# Autodesk Inventor assembly: Gripper Assembly
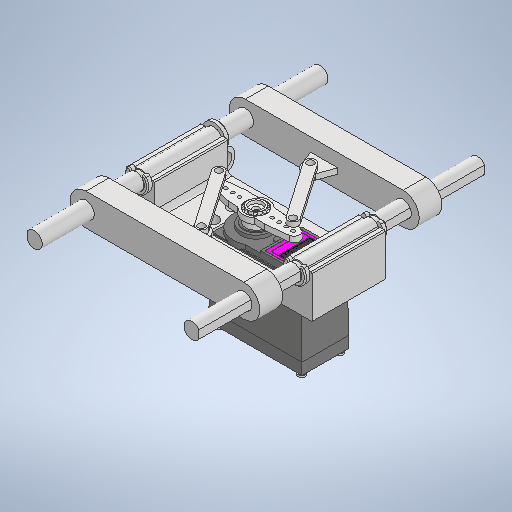
[picture p0: Inventor's stored thumbnail of the model, 512x512]
Saved by Autodesk Inventor 2025.2 (Build 292293000, 293)
## iProperties
Created: 2025-01-12
Part Number: Gripper Assembly
Document SubType Name: Assembly
Designer: caomi
Author: caomi
## Documents named in this file (8)
- C:\mnguyen\H2A\cad\Gripper\Gripper Assembly.iam
- C:\mnguyen\H2A\cad\Gripper\mg996R_v2\mg996R_v2\mg996R_v2.ipt
- C:\mnguyen\H2A\cad\Gripper\Servo mount - front.ipt
- C:\mnguyen\H2A\cad\Gripper\Linear Rod.ipt
- C:\mnguyen\H2A\cad\Gripper\Gripper_arms.ipt
- C:\mnguyen\H2A\cad\Gripper\Servo connector.ipt
- C:\mnguyen\H2A\cad\Gripper\Servo horn.ipt
- C:\mnguyen\H2A\cad\Gripper\C_clip.ipt
## Components (13 placed, 7 different names)
1. mg996R_v2:1 — Servo mount front - Servo, Servo horn - Servo
2. Servo mount - front:1 — Servo mount front - Servo, Linear Rod 1 - Servo mount front, Linear Rod 2 - Servo mount front
3. Linear Rod:1 — Linear Rod 1 - Servo mount front, Gripper arm 1 - Linear Rod 1, Gripper arm 2 - Linear Rod 1, Rigid:4, Rigid:5
4. Linear Rod:2 — Linear Rod 2 - Servo mount front, Gripper arm 1 - Linear Rod 2, Gripper arm 2 - Linear Rod 2, Rigid:7, Rigid:6
5. Gripper_arms:1 — Gripper arm 1 - Linear Rod 1, Gripper arm 1 - Linear Rod 2, Servo connector 1 - Gripper arm 1
6. Gripper_arms:2 — Gripper arm 2 - Linear Rod 1, Gripper arm 2 - Linear Rod 2, Servo connector 2 - Gripper arm 2
7. Servo connector:1 — Servo connector 1 - Gripper arm 1, Servo connector 1 - Servo horn
8. Servo horn:1 — Servo horn - Servo, Servo connector 1 - Servo horn, Servo connector 2 - Servo horn
9. Servo connector:2 — Servo connector 2 - Gripper arm 2, Servo connector 2 - Servo horn
10. C_clip:1 — Rigid:4
11. C_clip:2 — Rigid:5
12. C_clip:3 — Rigid:6
13. C_clip:4 — Rigid:7
## Relationships (16: WeldJoint 7, CylindricalJoint 6, RevoluteJoint 3)
- Servo mount front - Servo [WeldJoint]: mg996R_v2:1 ↔ Servo mount - front:1
- Linear Rod 1 - Servo mount front [WeldJoint]: Servo mount - front:1 ↔ Linear Rod:1
- Linear Rod 2 - Servo mount front [WeldJoint]: Servo mount - front:1 ↔ Linear Rod:2
- Gripper arm 1 - Linear Rod 1 [CylindricalJoint]: Linear Rod:1 ↔ Gripper_arms:1
- Gripper arm 1 - Linear Rod 2 [CylindricalJoint]: Linear Rod:2 ↔ Gripper_arms:1
- Gripper arm 2 - Linear Rod 1 [CylindricalJoint]: Linear Rod:1 ↔ Gripper_arms:2
- Gripper arm 2 - Linear Rod 2 [CylindricalJoint]: Linear Rod:2 ↔ Gripper_arms:2
- Servo connector 1 - Gripper arm 1 [RevoluteJoint]: Gripper_arms:1 ↔ Servo connector:1
- Servo horn - Servo [RevoluteJoint]: mg996R_v2:1 ↔ Servo horn:1
- Servo connector 1 - Servo horn [CylindricalJoint]: Servo connector:1 ↔ Servo horn:1
- Servo connector 2 - Gripper arm 2 [RevoluteJoint]: Gripper_arms:2 ↔ Servo connector:2
- Servo connector 2 - Servo horn [CylindricalJoint]: Servo horn:1 ↔ Servo connector:2
- Rigid:4 [WeldJoint]: Linear Rod:1 ↔ C_clip:1
- Rigid:5 [WeldJoint]: Linear Rod:1 ↔ C_clip:2
- Rigid:6 [WeldJoint]: Linear Rod:2 ↔ C_clip:3
- Rigid:7 [WeldJoint]: Linear Rod:2 ↔ C_clip:4
